# Autodesk Inventor assembly: MultiPass0V
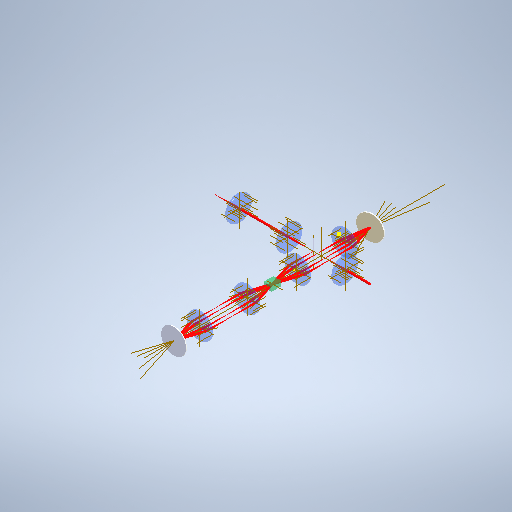
[picture p0: Inventor's stored thumbnail of the model, 512x512]
Saved by Autodesk Inventor 2025 (Build 290162010, 162A)
## iProperties
Created: 2024-08-19
Part Number: MultiPass0V
Document SubType Name: Assembly
Designer: User
Author: User
## Documents named in this file (13)
- C:\Users\User\Desktop\Hari_Laptop_Contents\KerlinLab\KTN\Multipass\MechanicalDrawing\MultiPass0V.iam
- C:\Users\User\Desktop\Hari_Laptop_Contents\KerlinLab\KTN\Multipass\MechanicalDrawing\BB1-E02-Solidworks.ipt
- C:\Users\User\Desktop\Hari_Laptop_Contents\KerlinLab\KTN\Multipass\MechanicalDrawing\LA1608-AB-Solidworks\LA1608-AB-Solidworks.ipt
- C:\Users\User\Desktop\Hari_Laptop_Contents\KerlinLab\KTN\Multipass\MechanicalDrawing\LaserBeamEntry1.ipt
- C:\Users\User\Desktop\Hari_Laptop_Contents\KerlinLab\KTN\Multipass\MechanicalDrawing\EntryMirror.ipt
- C:\Users\User\Desktop\Hari_Laptop_Contents\KerlinLab\KTN\Multipass\MechanicalDrawing\ExitMirror.ipt
- C:\Users\User\Desktop\Hari_Laptop_Contents\KerlinLab\KTN\Multipass\MechanicalDrawing\LaserBeamEntry2.ipt
- C:\Users\User\Desktop\Hari_Laptop_Contents\KerlinLab\KTN\Multipass\MechanicalDrawing\LaserBeamCenter1.ipt
- C:\Users\User\Desktop\Hari_Laptop_Contents\KerlinLab\KTN\Multipass\MechanicalDrawing\LaserBeamMirrorAngle1.ipt
- C:\Users\User\Desktop\Hari_Laptop_Contents\KerlinLab\KTN\Multipass\MechanicalDrawing\LaserBeamCenter2.ipt
- C:\Users\User\Desktop\Hari_Laptop_Contents\KerlinLab\KTN\Multipass\MechanicalDrawing\LaserBeamMirrorAngle2.ipt
- C:\Users\User\Desktop\Hari_Laptop_Contents\KerlinLab\KTN\Multipass\MechanicalDrawing\KTN1.ipt
- C:\Users\User\Desktop\Hari_Laptop_Contents\KerlinLab\KTN\Multipass\MechanicalDrawing\LoopPlane1.ipt
## Components (46 placed, 12 different names)
1. BB1-E02-Solidworks:1 — Mate:15, Mate:16, Mate:17, Mate:68, Mate:115, Mate:116, Mate:117
2. BB1-E02-Solidworks:2 — Mate:13, Mate:14, Mate:18, Mate:64, Mate:65, Mate:66, Mate:100, Mate:102
3. LA1608-AB-Solidworks:1 — Mate:5, Mate:6, Mate:7, Mate:8, Mate:11, Mate:12, Mate:45, Mate:48, Mate:50, Mate:53, Mate:55, Mate:56, Mate:72, Mate:78, Mate:80, Mate:81, Mate:86, Mate:88, Mate:106
4. LA1608-AB-Solidworks:3 — Mate:27, Mate:28, Mate:99, Mate:107, Mate:108
5. LA1608-AB-Solidworks:4 — Mate:7, Mate:8, Mate:12, Mate:13, Mate:14, Mate:18, Mate:49, Mate:51, Mate:52, Mate:54, Mate:73, Mate:77, Mate:79, Mate:82
6. LA1608-AB-Solidworks:5 — Mate:3, Mate:4, Mate:5, Mate:6, Mate:10, Mate:11, Mate:21, Mate:43, Flush:7, Mate:44, Mate:47, Mate:57, Mate:59, Mate:60, Mate:61, Mate:74, Mate:76, Mate:83, Mate:85, Mate:87, Mate:89, Mate:92, Flush:8, Mate:104, Mate:105
7. LA1608-AB-Solidworks:6 — Mate:3, Mate:4, Mate:10, Mate:15, Mate:16, Mate:17, Mate:19, Mate:20, Flush:1, Mate:33, Flush:5, Mate:38, Mate:41, Mate:42, Mate:63, Mate:75, Mate:84
8. LA1608-AB-Solidworks:7 — Mate:29, Flush:2, Mate:30, Mate:31, Flush:3
9. LaserBeamEntry1:1 — Mate:30, Mate:31
10. LaserBeamEntry1:2 — Mate:38, Flush:6, Mate:70
11. EntryMirror:1 — Mate:33, Mate:36, Flush:4
12. LaserBeamEntry2:1 — Mate:35, Flush:3
13. LaserBeamEntry2:2 — Mate:37, Flush:5, Flush:6
14. LaserBeamEntry2:3 — Mate:41, Mate:42
15. LaserBeamEntry2:4 — Mate:43, Flush:7
16. LaserBeamCenter1:1 — Mate:46, Mate:47
17. LaserBeamEntry2:5 — Mate:53, Mate:55
18. LaserBeamEntry2:6 — Mate:60, Mate:61, Mate:62
19. LaserBeamEntry2:8 — Mate:49, Mate:51
20. LaserBeamEntry2:9 — Mate:48, Mate:50
21. LaserBeamEntry2:10 — Mate:52, Mate:54
22. LaserBeamCenter1:2 — Mate:58, Mate:59
23. LaserBeamEntry2:11 — Mate:62, Mate:63
24. LaserBeamMirrorAngle1:1 — Mate:64, Mate:66, Mate:67, Mate:101
25. LaserBeamMirrorAngle1:2 — Mate:65, Mate:67
26. LaserBeamMirrorAngle1:3 — Mate:68, Mate:70, Mate:118
27. LaserBeamEntry2:12 — Mate:72, Mate:81
28. LaserBeamEntry2:13 — Mate:73, Mate:82
29. LaserBeamEntry2:14 — Mate:74, Mate:85
30. LaserBeamEntry2:15 — Mate:75, Mate:84
31. LaserBeamEntry2:16 — Mate:76, Mate:83
32. LaserBeamEntry2:17 — Mate:77, Mate:79
33. LaserBeamEntry2:18 — Mate:78, Mate:80, Mate:93
34. LaserBeamCenter2:1 — Mate:91, Mate:92
35. LaserBeamCenter2:2 — Mate:90, Mate:93
36. LaserBeamEntry2:19 — Mate:96, Mate:109
37. ExitMirror:2 — Mate:98, Mate:99, Flush:8
38. LaserBeamMirrorAngle2:1 — Mate:100, Mate:101, Mate:103
39. LaserBeamMirrorAngle2:2 — Mate:102, Mate:103
40. KTN1:1 — Mate:104, Mate:105, Mate:106, Mate:114
41. LA1608-AB-Solidworks:8 — Mate:107, Mate:108, Mate:110, Mate:112
42. LaserBeamCenter1:3 — Mate:109, Mate:110, Mate:111
43. LaserBeamEntry2:20 — Mate:111, Mate:112
44. LoopPlane1:1 — Mate:113, Mate:114
45. LaserBeamMirrorAngle2:3 — Mate:115, Mate:116
46. LaserBeamMirrorAngle1:4 — Mate:117, Mate:118
## Relationships (113: Mate 105, Flush 8)
- Mate:3: LA1608-AB-Solidworks:5 ↔ LA1608-AB-Solidworks:6
- Mate:4 (-50 mm): LA1608-AB-Solidworks:5 ↔ LA1608-AB-Solidworks:6
- Mate:5: LA1608-AB-Solidworks:1 ↔ LA1608-AB-Solidworks:5
- Mate:6 (50 mm): LA1608-AB-Solidworks:1 ↔ LA1608-AB-Solidworks:5
- Mate:7: LA1608-AB-Solidworks:1 ↔ LA1608-AB-Solidworks:4
- Mate:8 (-50 mm): LA1608-AB-Solidworks:1 ↔ LA1608-AB-Solidworks:4
- Mate:10: LA1608-AB-Solidworks:5 ↔ LA1608-AB-Solidworks:6
- Mate:11: LA1608-AB-Solidworks:1 ↔ LA1608-AB-Solidworks:5
- Mate:12: LA1608-AB-Solidworks:1 ↔ LA1608-AB-Solidworks:4
- Mate:13: BB1-E02-Solidworks:2 ↔ LA1608-AB-Solidworks:4
- Mate:14 (25 mm): BB1-E02-Solidworks:2 ↔ LA1608-AB-Solidworks:4
- Mate:15: BB1-E02-Solidworks:1 ↔ LA1608-AB-Solidworks:6
- Mate:16 (-25 mm): BB1-E02-Solidworks:1 ↔ LA1608-AB-Solidworks:6
- Mate:17: BB1-E02-Solidworks:1 ↔ LA1608-AB-Solidworks:6
- Mate:18: BB1-E02-Solidworks:2 ↔ LA1608-AB-Solidworks:4
- Mate:19: LA1608-AB-Solidworks:6
- Mate:20: LA1608-AB-Solidworks:6
- Mate:21: LA1608-AB-Solidworks:5
- Mate:22
- Mate:23
- Flush:1 (-25 mm): LA1608-AB-Solidworks:6
- Mate:24
- Mate:25
- Mate:27: LA1608-AB-Solidworks:3
- Mate:28 (-34 mm): LA1608-AB-Solidworks:3
- Mate:29: LA1608-AB-Solidworks:7
- Flush:2 (-25 mm): LA1608-AB-Solidworks:7
- Mate:30: LA1608-AB-Solidworks:7 ↔ LaserBeamEntry1:1
- Mate:31: LA1608-AB-Solidworks:7 ↔ LaserBeamEntry1:1
- Mate:33: LA1608-AB-Solidworks:6 ↔ EntryMirror:1
- Mate:35: LaserBeamEntry2:1
- Flush:3: LA1608-AB-Solidworks:7 ↔ LaserBeamEntry2:1
- Mate:36: EntryMirror:1
- Flush:4: EntryMirror:1
- Mate:37: LaserBeamEntry2:2
- Flush:5: LA1608-AB-Solidworks:6 ↔ LaserBeamEntry2:2
- Mate:38: LA1608-AB-Solidworks:6 ↔ LaserBeamEntry1:2
- Flush:6: LaserBeamEntry1:2 ↔ LaserBeamEntry2:2
- Mate:41: LA1608-AB-Solidworks:6 ↔ LaserBeamEntry2:3
- Mate:42: LA1608-AB-Solidworks:6 ↔ LaserBeamEntry2:3
- Mate:43: LA1608-AB-Solidworks:5 ↔ LaserBeamEntry2:4
- Flush:7: LA1608-AB-Solidworks:5 ↔ LaserBeamEntry2:4
- Mate:44: LA1608-AB-Solidworks:5
- Mate:45: LA1608-AB-Solidworks:1
- Mate:46: LaserBeamCenter1:1
- Mate:47: LA1608-AB-Solidworks:5 ↔ LaserBeamCenter1:1
- Mate:48: LA1608-AB-Solidworks:1 ↔ LaserBeamEntry2:9
- Mate:49: LA1608-AB-Solidworks:4 ↔ LaserBeamEntry2:8
- Mate:50: LA1608-AB-Solidworks:1 ↔ LaserBeamEntry2:9
- Mate:51: LA1608-AB-Solidworks:4 ↔ LaserBeamEntry2:8
- Mate:52: LA1608-AB-Solidworks:4 ↔ LaserBeamEntry2:10
- Mate:53: LA1608-AB-Solidworks:1 ↔ LaserBeamEntry2:5
- Mate:54: LA1608-AB-Solidworks:4 ↔ LaserBeamEntry2:10
- Mate:55: LA1608-AB-Solidworks:1 ↔ LaserBeamEntry2:5
- Mate:56: LA1608-AB-Solidworks:1
- Mate:57: LA1608-AB-Solidworks:5
- Mate:58: LaserBeamCenter1:2
- Mate:59: LA1608-AB-Solidworks:5 ↔ LaserBeamCenter1:2
- Mate:60: LA1608-AB-Solidworks:5 ↔ LaserBeamEntry2:6
- Mate:61: LA1608-AB-Solidworks:5 ↔ LaserBeamEntry2:6
- Mate:62: LaserBeamEntry2:6 ↔ LaserBeamEntry2:11
- Mate:63: LA1608-AB-Solidworks:6 ↔ LaserBeamEntry2:11
- Mate:64: BB1-E02-Solidworks:2 ↔ LaserBeamMirrorAngle1:1
- Mate:65: BB1-E02-Solidworks:2 ↔ LaserBeamMirrorAngle1:2
- Mate:66: BB1-E02-Solidworks:2 ↔ LaserBeamMirrorAngle1:1
- Mate:67: LaserBeamMirrorAngle1:1 ↔ LaserBeamMirrorAngle1:2
- Mate:68: BB1-E02-Solidworks:1 ↔ LaserBeamMirrorAngle1:3
- Mate:70: LaserBeamEntry1:2 ↔ LaserBeamMirrorAngle1:3
- Mate:72: LA1608-AB-Solidworks:1 ↔ LaserBeamEntry2:12
- Mate:73: LA1608-AB-Solidworks:4 ↔ LaserBeamEntry2:13
- Mate:74: LA1608-AB-Solidworks:5 ↔ LaserBeamEntry2:14
- Mate:75: LA1608-AB-Solidworks:6 ↔ LaserBeamEntry2:15
- Mate:76: LA1608-AB-Solidworks:5 ↔ LaserBeamEntry2:16
- Mate:77: LA1608-AB-Solidworks:4 ↔ LaserBeamEntry2:17
- Mate:78: LA1608-AB-Solidworks:1 ↔ LaserBeamEntry2:18
- Mate:79: LA1608-AB-Solidworks:4 ↔ LaserBeamEntry2:17
- Mate:80: LA1608-AB-Solidworks:1 ↔ LaserBeamEntry2:18
- Mate:81: LA1608-AB-Solidworks:1 ↔ LaserBeamEntry2:12
- Mate:82: LA1608-AB-Solidworks:4 ↔ LaserBeamEntry2:13
- Mate:83: LA1608-AB-Solidworks:5 ↔ LaserBeamEntry2:16
- Mate:84: LA1608-AB-Solidworks:6 ↔ LaserBeamEntry2:15
- Mate:85: LA1608-AB-Solidworks:5 ↔ LaserBeamEntry2:14
- Mate:86: LA1608-AB-Solidworks:1
- Mate:87: LA1608-AB-Solidworks:5
- Mate:88: LA1608-AB-Solidworks:1
- Mate:89: LA1608-AB-Solidworks:5
- Mate:90: LaserBeamCenter2:2
- Mate:91: LaserBeamCenter2:1
- Mate:92 (0.5 mm): LA1608-AB-Solidworks:5 ↔ LaserBeamCenter2:1
- Mate:93 (0.5 mm): LaserBeamEntry2:18 ↔ LaserBeamCenter2:2
- Mate:96: LaserBeamEntry2:19
- Mate:98: ExitMirror:2
- Mate:99: LA1608-AB-Solidworks:3 ↔ ExitMirror:2
- Flush:8: LA1608-AB-Solidworks:5 ↔ ExitMirror:2
- Mate:100: BB1-E02-Solidworks:2 ↔ LaserBeamMirrorAngle2:1
- Mate:101: LaserBeamMirrorAngle1:1 ↔ LaserBeamMirrorAngle2:1
- Mate:102: BB1-E02-Solidworks:2 ↔ LaserBeamMirrorAngle2:2
- Mate:103: LaserBeamMirrorAngle2:1 ↔ LaserBeamMirrorAngle2:2
- Mate:104: LA1608-AB-Solidworks:5 ↔ KTN1:1
- Mate:105 (25 mm): LA1608-AB-Solidworks:5 ↔ KTN1:1
- Mate:106: LA1608-AB-Solidworks:1 ↔ KTN1:1
- Mate:107: LA1608-AB-Solidworks:3 ↔ LA1608-AB-Solidworks:8
- Mate:108 (50 mm): LA1608-AB-Solidworks:3 ↔ LA1608-AB-Solidworks:8
- Mate:109: LaserBeamEntry2:19 ↔ LaserBeamCenter1:3
- Mate:110: LA1608-AB-Solidworks:8 ↔ LaserBeamCenter1:3
- Mate:111: LaserBeamCenter1:3 ↔ LaserBeamEntry2:20
- Mate:112: LA1608-AB-Solidworks:8 ↔ LaserBeamEntry2:20
- Mate:113: LoopPlane1:1
- Mate:114: KTN1:1 ↔ LoopPlane1:1
- Mate:115: BB1-E02-Solidworks:1 ↔ LaserBeamMirrorAngle2:3
- Mate:116: BB1-E02-Solidworks:1 ↔ LaserBeamMirrorAngle2:3
- Mate:117: BB1-E02-Solidworks:1 ↔ LaserBeamMirrorAngle1:4
- Mate:118: LaserBeamMirrorAngle1:3 ↔ LaserBeamMirrorAngle1:4
